# Autodesk Inventor assembly: 部件1
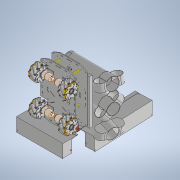
[picture p0: Inventor's stored thumbnail of the model, 180x180]
Saved by Autodesk Inventor 2020 (Build 240168000, 168)
## iProperties
Created: 2020-12-02
Part Number: 部件1
Document SubType Name: Assembly
Designer: huang
Author: huang
## Documents named in this file (18)
- C:\Users\huang\Desktop\车\部件1.iam
- C:\Users\huang\Desktop\车\底板2.ipt
- C:\Users\huang\Desktop\车\马达固定.ipt
- C:\Users\huang\Desktop\车\Moteur DC encodeur\Moteur DC encodeur.iam
- C:\Users\huang\Desktop\车\100mm Aluminum Mecanum wheels\100mm Aluminum Mecanum wheels.iam
- C:\Users\huang\Desktop\车\六角长螺母.ipt
- C:\Users\huang\Desktop\车\底板1.ipt
- C:\Users\huang\Desktop\车\滑轨.ipt
- C:\Users\huang\Desktop\车\滑轨座.ipt
- C:\Users\huang\Desktop\车\固定架.ipt
- C:\Users\huang\Desktop\车\回收桶.ipt
- C:\Users\huang\Desktop\车\角度.ipt
- C:\Users\huang\Desktop\车\servo-pwm-control-1.snapshot.13\DIGITAL SERVO ASSEMBLY.iam
- C:\Users\huang\Desktop\车\零件1.ipt
- C:\Users\huang\Desktop\车\22.ipt
- C:\Users\huang\Desktop\车\零件.ipt
- C:\Users\huang\Desktop\车\servo-pwm-control-1.snapshot.13\Servo Arm for DS3218MG.ipt
- D:\学校\3D打印\新建文件夹 (2)\零件1.ipt
## Components (38 placed, 16 different names)
1. 底板2:1 — 插入:1, 插入:2, 插入:3, 插入:4, 插入:5, 插入:6, 插入:7, 插入:8, 插入:23, 插入:24, 插入:25, 插入:26, 插入:27, 插入:28, 配合:2, 插入:64, 配合:3
2. 马达固定:1 — 插入:1, 插入:2, 插入:11, 插入:12
3. 马达固定:2 — 插入:3, 插入:4, 插入:9, 插入:10
4. 马达固定:3 — 插入:5, 插入:6, 插入:15, 插入:16
5. 马达固定:4 — 插入:7, 插入:8, 插入:13, 插入:14
6. Moteur DC encodeur:1 [sub-assembly] — 插入:9, 插入:10, 插入:17
7. Moteur DC encodeur:2 [sub-assembly] — 插入:11, 插入:12, 插入:19
8. Moteur DC encodeur:3 [sub-assembly] — 插入:15, 插入:16, 插入:18
9. Moteur DC encodeur:4 [sub-assembly] — 插入:13, 插入:14, 插入:20
10. 100mm Aluminum Mecanum wheels:1 [sub-assembly] — 插入:17
11. 100mm Aluminum Mecanum wheels:2 [sub-assembly] — 插入:18
12. 100mm Aluminum Mecanum wheels:3 [sub-assembly] — 插入:19
13. 100mm Aluminum Mecanum wheels:4 [sub-assembly] — 插入:20
14. 六角长螺母:2 — 插入:24, 插入:34
15. 六角长螺母:4 — 插入:23
16. 六角长螺母:5 — 插入:25
17. 六角长螺母:6 — 插入:26
18. 六角长螺母:7 — 插入:27, 插入:33
19. 六角长螺母:8 — 插入:28
20. 底板1:1 — 插入:31, 插入:32, 插入:33, 插入:34
21. 滑轨:1 — 插入:31, 插入:32, 圆柱:1, 圆柱:2
22. 滑轨座:1 — 圆柱:1, 圆柱:2, 插入:35, 插入:36
23. 固定架:1 — 插入:35, 插入:36, 插入:37, 插入:38, 插入:40, 插入:41, 插入:42, 插入:43
24. 角度:1 — 插入:37, 插入:38, 插入:57
25. 回收桶:1 — 插入:53, 插入:57
26. 角度:2 — 插入:40, 插入:41, 插入:56
27. 角度:3 — 插入:42, 插入:43, 插入:58
28. 回收桶:2 — 插入:55, 插入:56
29. 回收桶:3 — 插入:54, 插入:58
30. DIGITAL SERVO ASSEMBLY:1 [sub-assembly] — 插入:50, 插入:65, 插入:66
31. 零件1:1 — 配合:2
32. Servo Arm for DS3218MG:1 — 插入:50, 插入:62, 插入:63
33. 22:1 — 插入:62, 插入:63
34. 零件1:2 — 插入:53
35. 零件1:3 — 插入:54
36. 零件1:4 — 插入:55
37. 零件:2 — 插入:64, 插入:66
38. 零件:3 — 配合:3, 插入:65
## Relationships (54: Insert 50, CylindricalJoint 2, Mate 2)
- 插入:1 [Insert]: 底板2:1 ↔ 马达固定:1
- 插入:2 [Insert]: 底板2:1 ↔ 马达固定:1
- 插入:3 [Insert]: 底板2:1 ↔ 马达固定:2
- 插入:4 [Insert]: 底板2:1 ↔ 马达固定:2
- 插入:5 [Insert]: 底板2:1 ↔ 马达固定:3
- 插入:6 [Insert]: 底板2:1 ↔ 马达固定:3
- 插入:7 [Insert]: 底板2:1 ↔ 马达固定:4
- 插入:8 [Insert]: 底板2:1 ↔ 马达固定:4
- 插入:9 [Insert]: 马达固定:2 ↔ Moteur DC encodeur:1
- 插入:10 [Insert]: 马达固定:2 ↔ Moteur DC encodeur:1
- 插入:11 [Insert]: 马达固定:1 ↔ Moteur DC encodeur:2
- 插入:12 [Insert]: 马达固定:1 ↔ Moteur DC encodeur:2
- 插入:13 [Insert]: 马达固定:4 ↔ Moteur DC encodeur:4
- 插入:14 [Insert]: 马达固定:4 ↔ Moteur DC encodeur:4
- 插入:15 [Insert]: 马达固定:3 ↔ Moteur DC encodeur:3
- 插入:16 [Insert]: 马达固定:3 ↔ Moteur DC encodeur:3
- 插入:17 [Insert]: Moteur DC encodeur:1 ↔ 100mm Aluminum Mecanum wheels:1
- 插入:18 [Insert]: Moteur DC encodeur:3 ↔ 100mm Aluminum Mecanum wheels:2
- 插入:19 [Insert]: Moteur DC encodeur:2 ↔ 100mm Aluminum Mecanum wheels:3
- 插入:20 [Insert]: Moteur DC encodeur:4 ↔ 100mm Aluminum Mecanum wheels:4
- 插入:23 [Insert]: 底板2:1 ↔ 六角长螺母:4
- 插入:24 [Insert]: 底板2:1 ↔ 六角长螺母:2
- 插入:25 [Insert]: 底板2:1 ↔ 六角长螺母:5
- 插入:26 [Insert]: 底板2:1 ↔ 六角长螺母:6
- 插入:27 [Insert]: 底板2:1 ↔ 六角长螺母:7
- 插入:28 [Insert]: 底板2:1 ↔ 六角长螺母:8
- 插入:31 [Insert]: 底板1:1 ↔ 滑轨:1
- 插入:32 [Insert]: 底板1:1 ↔ 滑轨:1
- 圆柱:1 [CylindricalJoint]: 滑轨:1 ↔ 滑轨座:1
- 圆柱:2 [CylindricalJoint]: 滑轨:1 ↔ 滑轨座:1
- 插入:33 [Insert]: 六角长螺母:7 ↔ 底板1:1
- 插入:34 [Insert]: 六角长螺母:2 ↔ 底板1:1
- 插入:35 [Insert]: 滑轨座:1 ↔ 固定架:1
- 插入:36 [Insert]: 滑轨座:1 ↔ 固定架:1
- 插入:37 [Insert]: 固定架:1 ↔ 角度:1
- 插入:38 [Insert]: 固定架:1 ↔ 角度:1
- 插入:40 [Insert]: 固定架:1 ↔ 角度:2
- 插入:41 [Insert]: 固定架:1 ↔ 角度:2
- 插入:42 [Insert]: 固定架:1 ↔ 角度:3
- 插入:43 [Insert]: 固定架:1 ↔ 角度:3
- 配合:2 [Mate]: 底板2:1 ↔ 零件1:1
- 插入:50 [Insert]: DIGITAL SERVO ASSEMBLY:1 ↔ Servo Arm for DS3218MG:1
- 插入:53 [Insert]: 回收桶:1 ↔ 零件1:2
- 插入:54 [Insert]: 回收桶:3 ↔ 零件1:3
- 插入:55 [Insert]: 回收桶:2 ↔ 零件1:4
- 插入:56 [Insert] (-10 mm): 角度:2 ↔ 回收桶:2
- 插入:57 [Insert] (-10 mm): 角度:1 ↔ 回收桶:1
- 插入:58 [Insert] (-10 mm): 角度:3 ↔ 回收桶:3
- 插入:62 [Insert]: Servo Arm for DS3218MG:1 ↔ 22:1
- 插入:63 [Insert]: Servo Arm for DS3218MG:1 ↔ 22:1
- 插入:64 [Insert]: 底板2:1 ↔ 零件:2
- 配合:3 [Mate]: 底板2:1 ↔ 零件:3
- 插入:65 [Insert]: DIGITAL SERVO ASSEMBLY:1 ↔ 零件:3
- 插入:66 [Insert]: DIGITAL SERVO ASSEMBLY:1 ↔ 零件:2
